# Autodesk Inventor assembly: launcher.mainAssembly
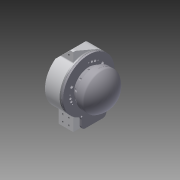
[picture p0: Inventor's stored thumbnail of the model, 180x180]
Saved by Autodesk Inventor 2011 (Build 150239000, 239)
## iProperties
Created: 2011-02-22
Part Number: launcher.mainAssembly
Document SubType Name: Assembly
Designer: Casey
Author: Casey
## Documents named in this file (7)
- C:\Users\M. Woods III\Desktop\design\Mechanical Drawings\launcher_1.iam
- C:\Users\M. Woods III\Desktop\design\Mechanical Drawings\launcher_1_housing.ipt
- C:\Users\M. Woods III\Desktop\design\Mechanical Drawings\capsule.iam
- C:\Users\M. Woods III\Desktop\design\Mechanical Drawings\launcher_3x8x4_bearing.ipt
- C:\Users\M. Woods III\Desktop\design\Mechanical Drawings\launcher_1_cap.ipt
- C:\Users\M. Woods III\Desktop\design\Mechanical Drawings\launcher_cam.ipt
- C:\Users\M. Woods III\Desktop\design\Mechanical Drawings\launcher_latch.ipt
## Components (16 placed, 6 different names)
1. launcher_1_housing:1 — Mate:7, Tangent:5, Mate:8, Mate:9, Mate:10, Mate:11, Mate:12, Mate:13, Flush:5, Mate:14, Mate:15, Mate:16, Flush:7, Mate:17, Mate:18, Mate:19, Mate:24, Mate:25, Mate:26
2. capsule:1 [sub-assembly] — Mate:7, Tangent:5
3. launcher_3x8x4_bearing:1 — Mate:13, Flush:2, Flush:3
4. launcher_3x8x4_bearing:2 — Mate:12, Flush:2, Flush:4
5. launcher_3x8x4_bearing:3 — Mate:11, Flush:4, Flush:6
6. launcher_3x8x4_bearing:4 — Mate:10, Flush:6
7. launcher_3x8x4_bearing:5 — Mate:9, Flush:1, Flush:5
8. launcher_3x8x4_bearing:6 — Mate:8, Flush:1, Flush:3
9. launcher_3x8x4_bearing:7 — Mate:14, Flush:7, Flush:8
10. launcher_3x8x4_bearing:8 — Mate:15, Flush:9
11. launcher_3x8x4_bearing:9 — Mate:16, Flush:8, Flush:9, Mate:23
12. launcher_1_cap:1 — Mate:17, Mate:18, Mate:19
13. launcher_cam:1 — Mate:25, Mate:26
14. launcher_latch:1 — Mate:23, Mate:24
15. launcher_latch:2
16. launcher_latch:3
## Component patterns: (3 elements, first: launcher_latch:1)
## Relationships (27: Mate 17, Flush 9, Tangent 1)
- Mate:7: launcher_1_housing:1 ↔ capsule:1
- Tangent:5: launcher_1_housing:1 ↔ capsule:1
- Mate:8: launcher_1_housing:1 ↔ launcher_3x8x4_bearing:6
- Mate:9: launcher_1_housing:1 ↔ launcher_3x8x4_bearing:5
- Mate:10: launcher_1_housing:1 ↔ launcher_3x8x4_bearing:4
- Mate:11: launcher_1_housing:1 ↔ launcher_3x8x4_bearing:3
- Mate:12: launcher_1_housing:1 ↔ launcher_3x8x4_bearing:2
- Mate:13: launcher_1_housing:1 ↔ launcher_3x8x4_bearing:1
- Flush:1: launcher_3x8x4_bearing:5 ↔ launcher_3x8x4_bearing:6
- Flush:2: launcher_3x8x4_bearing:1 ↔ launcher_3x8x4_bearing:2
- Flush:3: launcher_3x8x4_bearing:1 ↔ launcher_3x8x4_bearing:6
- Flush:4: launcher_3x8x4_bearing:2 ↔ launcher_3x8x4_bearing:3
- Flush:5: launcher_1_housing:1 ↔ launcher_3x8x4_bearing:5
- Flush:6: launcher_3x8x4_bearing:3 ↔ launcher_3x8x4_bearing:4
- Mate:14: launcher_1_housing:1 ↔ launcher_3x8x4_bearing:7
- Mate:15: launcher_1_housing:1 ↔ launcher_3x8x4_bearing:8
- Mate:16: launcher_1_housing:1 ↔ launcher_3x8x4_bearing:9
- Flush:7: launcher_1_housing:1 ↔ launcher_3x8x4_bearing:7
- Flush:8: launcher_3x8x4_bearing:7 ↔ launcher_3x8x4_bearing:9
- Flush:9: launcher_3x8x4_bearing:8 ↔ launcher_3x8x4_bearing:9
- Mate:17: launcher_1_housing:1 ↔ launcher_1_cap:1
- Mate:18: launcher_1_housing:1 ↔ launcher_1_cap:1
- Mate:19: launcher_1_housing:1 ↔ launcher_1_cap:1
- Mate:23: launcher_3x8x4_bearing:9 ↔ launcher_latch:1
- Mate:24: launcher_1_housing:1 ↔ launcher_latch:1
- Mate:25: launcher_1_housing:1 ↔ launcher_cam:1
- Mate:26: launcher_1_housing:1 ↔ launcher_cam:1
